# Autodesk Inventor assembly: gakutasu-cat-wheel
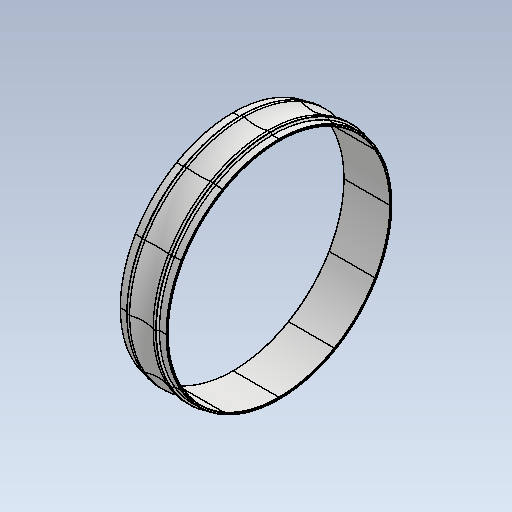
[picture p0: Inventor's stored thumbnail of the model, 512x512]
Saved by Autodesk Inventor 2026.2 (Build 302298000, 298)
## iProperties
Created: 2026-01-17
Part Number: gakutasu-cat-wheel
Document SubType Name: Assembly
Designer: gakut
Author: gakut
## Documents named in this file (3)
- C:\Users\gakut\Documents\Inventor\gakutasu-cat-wheel\gakutasu-cat-wheel.iam
- C:\Users\gakut\Documents\Inventor\gakutasu-cat-wheel\parts\wheel_plate.ipt
- C:\Users\gakut\Documents\Inventor\gakutasu-cat-wheel\parts\plate_joint_shaft.ipt
## Components (13 placed, 2 different names)
1. wheel_plate:1 — Mate:1, Flush:1, Rigid:1
2. wheel_plate:2 — Rigid:1, Rigid:3
3. wheel_plate:3 — Rigid:3
4. wheel_plate:4 — Rigid:9
5. wheel_plate:5 — Rigid:9
6. wheel_plate:6 — Rigid:10
7. wheel_plate:7 — Rigid:10
8. wheel_plate:8
9. wheel_plate:9
10. wheel_plate:10 — Rigid:11
11. wheel_plate:11 — Rigid:11
12. wheel_plate:12
13. plate_joint_shaft:1 — Mate:1, Flush:1
## Relationships (13: WeldJoint 11, Mate 1, Flush 1)
- Mate:1: wheel_plate:1 ↔ plate_joint_shaft:1
- Flush:1: wheel_plate:1 ↔ plate_joint_shaft:1
- Rigid:1 [WeldJoint]: wheel_plate:1 ↔ wheel_plate:2
- [WeldJoint]: wheel_plate:3 ↔ wheel_plate:4
- Rigid:3 [WeldJoint]: wheel_plate:2 ↔ wheel_plate:3
- [WeldJoint]: wheel_plate:5 ↔ wheel_plate:6
- Rigid:9 [WeldJoint]: wheel_plate:4 ↔ wheel_plate:5
- [WeldJoint]: wheel_plate:7 ↔ wheel_plate:8
- [WeldJoint]: wheel_plate:9 ↔ wheel_plate:10
- [WeldJoint]: wheel_plate:8 ↔ wheel_plate:9
- [WeldJoint]: wheel_plate:11 ↔ wheel_plate:12
- Rigid:11 [WeldJoint]: wheel_plate:10 ↔ wheel_plate:11
- Rigid:10 [WeldJoint]: wheel_plate:6 ↔ wheel_plate:7
## Named parameters: d17_d16 = 0 mm, d19_d17_d16 = 0 mm, d22_d19_d17_d16 = 0 mm, d23_d20 = 0 mm, d24_d21 = 162.214152 deg, d25_d16 = 0 mm, d26_d17_d16 = 0 mm, d27_d18 = 0 mm
